# Autodesk Inventor assembly: frontBackFacing
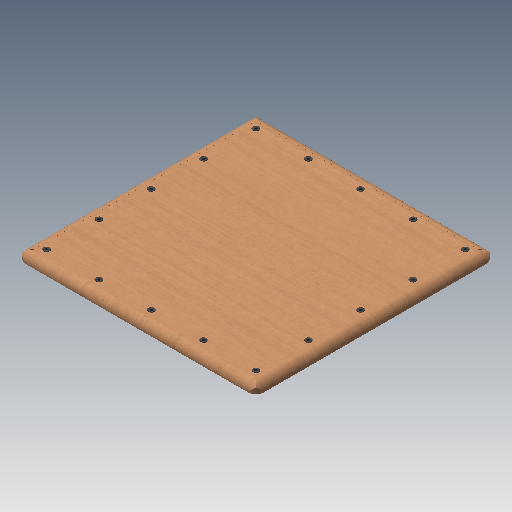
[picture p0: Inventor's stored thumbnail of the model, 512x512]
Saved by Autodesk Inventor 2018.2 (Build 222227000, 227)
## iProperties
Created: 2016-04-01
Part Number: frontBackFacing
Document SubType Name: Assembly
Designer: sawai
Author: sawai
## Documents named in this file (6)
- C:\Users\sawaiz\OneDrive\projects\modularRICHFrame\facing\frontBackFacing.iam
- C:\Users\sawaiz\OneDrive\projects\modularRICHFrame\facing\frontBackFace.ipt
- C:\Users\sawaiz\OneDrive\projects\modularRICHFrame\facing\frontBackMoulding.ipt
- C:\Users\sawaiz\OneDrive\projects\modularRICHFrame\facing\frontBackGasket.ipt
- C:\Users\sawaiz\OneDrive\projects\modularRICHFrame\hardware\m5x12BlackSocketHead.ipt
- C:\Users\sawaiz\OneDrive\projects\modularRICHFrame\hardware\m5TNut.ipt
## Components (34 placed, 5 different names)
1. frontBackFace:1 — Mate:1, Mate:2, Mate:3, Mate:4, Mate:8, Mate:9, Mate:10, Mate:13, Flush:6, Mate:14, Flush:7, Angle:1
2. frontBackMoulding:1 — Mate:1, Mate:5, Mate:6, Flush:3, Flush:4, Flush:5, Mate:11, Mate:12
3. frontBackMoulding:2 — Mate:2, Mate:5, Mate:7, Flush:1, Flush:4, Mate:11, Mate:12
4. frontBackMoulding:3 — Mate:4, Mate:6, Flush:2, Flush:3
5. frontBackMoulding:4 — Mate:3, Mate:7, Flush:1, Flush:2
6. frontBackGasket:1 — Mate:8, Mate:9, Mate:10, Flush:5, Mate:16
7. m5x12BlackSocketHead:1 — Mate:13, Flush:6
8. m5x12BlackSocketHead:2
9. m5x12BlackSocketHead:3
10. m5x12BlackSocketHead:4
11. m5x12BlackSocketHead:5
12. m5x12BlackSocketHead:6
13. m5x12BlackSocketHead:7
14. m5x12BlackSocketHead:8
15. m5x12BlackSocketHead:9
16. m5x12BlackSocketHead:10
17. m5x12BlackSocketHead:11 — Mate:14, Flush:7, Mate:15
18. m5x12BlackSocketHead:12
19. m5x12BlackSocketHead:13
20. m5x12BlackSocketHead:14
21. m5x12BlackSocketHead:15
22. m5x12BlackSocketHead:16
23. m5TNut:1 — Mate:15, Angle:1, Mate:16
24. m5TNut:2
25. m5TNut:3
26. m5TNut:4
27. m5TNut:5
28. m5TNut:6
29. m5TNut:7
30. m5TNut:8
31. m5TNut:9
32. m5TNut:10
33. m5TNut:11
34. m5TNut:12
## Component patterns: (10 elements, first: m5x12BlackSocketHead:1), (6 elements, first: m5x12BlackSocketHead:11), (4 elements), (3 elements, first: m5TNut:1), Component Pattern 3:2 (3 elements), Component Pattern 3:3 (3 elements), Component Pattern 3:4 (3 elements)
## Relationships (24: Mate 16, Flush 7, Angle 1)
- Mate:1: frontBackFace:1 ↔ frontBackMoulding:1
- Mate:2: frontBackFace:1 ↔ frontBackMoulding:2
- Mate:3: frontBackFace:1 ↔ frontBackMoulding:4
- Mate:4: frontBackFace:1 ↔ frontBackMoulding:3
- Mate:5: frontBackMoulding:1 ↔ frontBackMoulding:2
- Mate:6: frontBackMoulding:1 ↔ frontBackMoulding:3
- Mate:7: frontBackMoulding:2 ↔ frontBackMoulding:4
- Flush:1: frontBackMoulding:2 ↔ frontBackMoulding:4
- Flush:2: frontBackMoulding:3 ↔ frontBackMoulding:4
- Flush:3: frontBackMoulding:1 ↔ frontBackMoulding:3
- Flush:4: frontBackMoulding:1 ↔ frontBackMoulding:2
- Mate:8: frontBackFace:1 ↔ frontBackGasket:1
- Mate:9: frontBackFace:1 ↔ frontBackGasket:1
- Mate:10: frontBackFace:1 ↔ frontBackGasket:1
- Flush:5: frontBackMoulding:1 ↔ frontBackGasket:1
- Mate:11: frontBackMoulding:1 ↔ frontBackMoulding:2
- Mate:12: frontBackMoulding:1 ↔ frontBackMoulding:2
- Mate:13: frontBackFace:1 ↔ m5x12BlackSocketHead:1
- Flush:6: frontBackFace:1 ↔ m5x12BlackSocketHead:1
- Mate:14: frontBackFace:1 ↔ m5x12BlackSocketHead:11
- Flush:7: frontBackFace:1 ↔ m5x12BlackSocketHead:11
- Mate:15: m5x12BlackSocketHead:11 ↔ m5TNut:1
- Angle:1 (0 deg): frontBackFace:1 ↔ m5TNut:1
- Mate:16 (2 mm): frontBackGasket:1 ↔ m5TNut:1
